# Autodesk Inventor assembly: Controller Asssembly
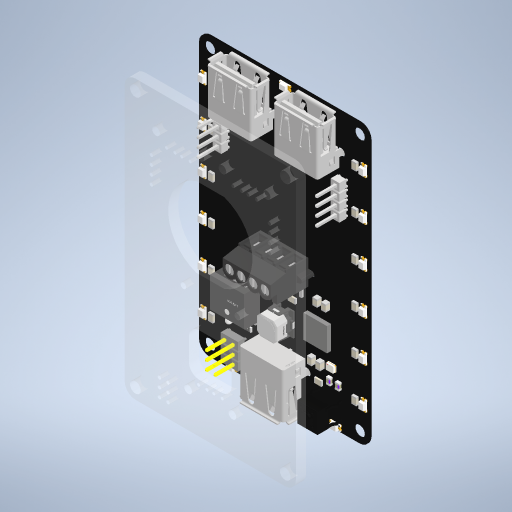
[picture p0: Inventor's stored thumbnail of the model, 512x512]
Saved by Autodesk Inventor 2023 (Build 270158000, 158)
## iProperties
Created: 2022-08-29
Part Number: Controller Asssembly
Document SubType Name: Assembly
Designer: swift
Author: swift
## Documents named in this file (3)
- C:\Users\swift\workspace\Fairy Light Controller\Controller Cover\Controller Asssembly.iam
- C:\Users\swift\workspace\Fairy Light Controller\Controller Cover\Fairy_Light_Controller_PCB_v1.ipt
- C:\Users\swift\workspace\Fairy Light Controller\Controller Cover\Cover.ipt
## Components (2 placed, 2 different names)
1. Fairy_Light_Controller_PCB_v1:1 — Mate:1
2. Cover:1 — Mate:1
## Relationships (1: Mate 1)
- Mate:1 (19.05 mm): Fairy_Light_Controller_PCB_v1:1 ↔ Cover:1
